# Autodesk Inventor assembly: Combined OmniWheel
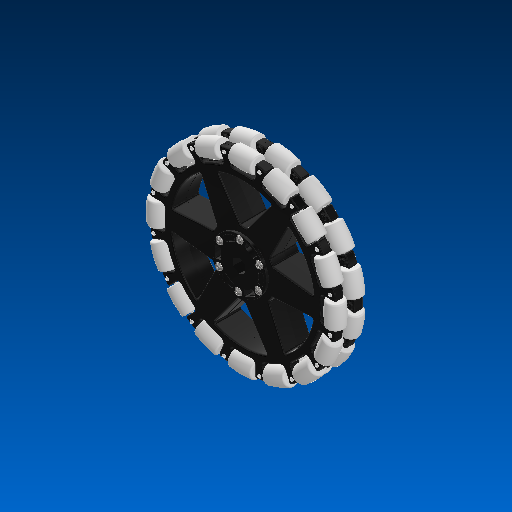
[picture p0: Inventor's stored thumbnail of the model, 512x512]
Saved by Autodesk Inventor 2022.2 (Build 262287000, 287)
## iProperties
Created: 2022-01-02
Part Number: Combined OmniWheel
Document SubType Name: Assembly
Designer: omard
Author: omard
## Documents named in this file (4)
- D:\omard\OneDrive - Auburn University\BasketBall Shooting Robot\Combined OmniWheel.iam
- D:\omard\OneDrive - Auburn University\BasketBall Shooting Robot\VEX Parts\1_2” Hex Bore Aluminum VersaHub (217-2592).ipt
- D:\omard\OneDrive - Auburn University\BasketBall Shooting Robot\VEX Parts\8 Omni-Directional Wheel (217-2613).iam
- D:\omard\OneDrive - Auburn University\BasketBall Shooting Robot\VEX Parts\#8-32 x 0.625 Star Drive Screw (276-4993).ipt
## Components (15 placed, 3 different names)
1. 1_2” Hex Bore Aluminum VersaHub (217-2592):1 — Mate:1, Mate:2, Mate:3, Angle:1, Mate:19, Mate:20, Mate:21, Mate:22, Mate:23, Mate:24, Mate:25, Mate:26, Mate:27, Mate:28, Mate:29, Mate:30
2. 8 Omni-Directional Wheel (217-2613):1 [sub-assembly] — Mate:1, Mate:2, Mate:3, Angle:1, Angle:2, Mate:4, Mate:5, Mate:6
3. 1_2” Hex Bore Aluminum VersaHub (217-2592):2 — Angle:2, Mate:4, Mate:5, Mate:6, Mate:7, Mate:8, Mate:9, Mate:10, Mate:11, Mate:12, Mate:13, Mate:14, Mate:15, Mate:16, Mate:17, Mate:18
4. #8-32 x 0.625 Star Drive Screw (276-4993):1 — Mate:7, Mate:14
5. #8-32 x 0.625 Star Drive Screw (276-4993):2 — Mate:12, Mate:13
6. #8-32 x 0.625 Star Drive Screw (276-4993):3 — Mate:11, Mate:18
7. #8-32 x 0.625 Star Drive Screw (276-4993):4 — Mate:10, Mate:17
8. #8-32 x 0.625 Star Drive Screw (276-4993):5 — Mate:9, Mate:16
9. #8-32 x 0.625 Star Drive Screw (276-4993):6 — Mate:8, Mate:15
10. #8-32 x 0.625 Star Drive Screw (276-4993):7 — Mate:25, Mate:30
11. #8-32 x 0.625 Star Drive Screw (276-4993):8 — Mate:24, Mate:29
12. #8-32 x 0.625 Star Drive Screw (276-4993):9 — Mate:23, Mate:28
13. #8-32 x 0.625 Star Drive Screw (276-4993):10 — Mate:22, Mate:27
14. #8-32 x 0.625 Star Drive Screw (276-4993):11 — Mate:19, Mate:20
15. #8-32 x 0.625 Star Drive Screw (276-4993):12 — Mate:21, Mate:26
## Relationships (32: Mate 30, Angle 2)
- Mate:1: 1_2” Hex Bore Aluminum VersaHub (217-2592):1 ↔ 8 Omni-Directional Wheel (217-2613):1
- Mate:2: 1_2” Hex Bore Aluminum VersaHub (217-2592):1 ↔ 8 Omni-Directional Wheel (217-2613):1
- Mate:3: 1_2” Hex Bore Aluminum VersaHub (217-2592):1 ↔ 8 Omni-Directional Wheel (217-2613):1
- Angle:1 (0 deg): 1_2” Hex Bore Aluminum VersaHub (217-2592):1 ↔ 8 Omni-Directional Wheel (217-2613):1
- Angle:2 (0 deg): 8 Omni-Directional Wheel (217-2613):1 ↔ 1_2” Hex Bore Aluminum VersaHub (217-2592):2
- Mate:4: 8 Omni-Directional Wheel (217-2613):1 ↔ 1_2” Hex Bore Aluminum VersaHub (217-2592):2
- Mate:5: 8 Omni-Directional Wheel (217-2613):1 ↔ 1_2” Hex Bore Aluminum VersaHub (217-2592):2
- Mate:6: 8 Omni-Directional Wheel (217-2613):1 ↔ 1_2” Hex Bore Aluminum VersaHub (217-2592):2
- Mate:7: 1_2” Hex Bore Aluminum VersaHub (217-2592):2 ↔ #8-32 x 0.625 Star Drive Screw (276-4993):1
- Mate:8: 1_2” Hex Bore Aluminum VersaHub (217-2592):2 ↔ #8-32 x 0.625 Star Drive Screw (276-4993):6
- Mate:9: 1_2” Hex Bore Aluminum VersaHub (217-2592):2 ↔ #8-32 x 0.625 Star Drive Screw (276-4993):5
- Mate:10: 1_2” Hex Bore Aluminum VersaHub (217-2592):2 ↔ #8-32 x 0.625 Star Drive Screw (276-4993):4
- Mate:11: 1_2” Hex Bore Aluminum VersaHub (217-2592):2 ↔ #8-32 x 0.625 Star Drive Screw (276-4993):3
- Mate:12: 1_2” Hex Bore Aluminum VersaHub (217-2592):2 ↔ #8-32 x 0.625 Star Drive Screw (276-4993):2
- Mate:13: 1_2” Hex Bore Aluminum VersaHub (217-2592):2 ↔ #8-32 x 0.625 Star Drive Screw (276-4993):2
- Mate:14: 1_2” Hex Bore Aluminum VersaHub (217-2592):2 ↔ #8-32 x 0.625 Star Drive Screw (276-4993):1
- Mate:15: 1_2” Hex Bore Aluminum VersaHub (217-2592):2 ↔ #8-32 x 0.625 Star Drive Screw (276-4993):6
- Mate:16: 1_2” Hex Bore Aluminum VersaHub (217-2592):2 ↔ #8-32 x 0.625 Star Drive Screw (276-4993):5
- Mate:17: 1_2” Hex Bore Aluminum VersaHub (217-2592):2 ↔ #8-32 x 0.625 Star Drive Screw (276-4993):4
- Mate:18: 1_2” Hex Bore Aluminum VersaHub (217-2592):2 ↔ #8-32 x 0.625 Star Drive Screw (276-4993):3
- Mate:19: 1_2” Hex Bore Aluminum VersaHub (217-2592):1 ↔ #8-32 x 0.625 Star Drive Screw (276-4993):11
- Mate:20: 1_2” Hex Bore Aluminum VersaHub (217-2592):1 ↔ #8-32 x 0.625 Star Drive Screw (276-4993):11
- Mate:21: 1_2” Hex Bore Aluminum VersaHub (217-2592):1 ↔ #8-32 x 0.625 Star Drive Screw (276-4993):12
- Mate:22: 1_2” Hex Bore Aluminum VersaHub (217-2592):1 ↔ #8-32 x 0.625 Star Drive Screw (276-4993):10
- Mate:23: 1_2” Hex Bore Aluminum VersaHub (217-2592):1 ↔ #8-32 x 0.625 Star Drive Screw (276-4993):9
- Mate:24: 1_2” Hex Bore Aluminum VersaHub (217-2592):1 ↔ #8-32 x 0.625 Star Drive Screw (276-4993):8
- Mate:25: 1_2” Hex Bore Aluminum VersaHub (217-2592):1 ↔ #8-32 x 0.625 Star Drive Screw (276-4993):7
- Mate:26: 1_2” Hex Bore Aluminum VersaHub (217-2592):1 ↔ #8-32 x 0.625 Star Drive Screw (276-4993):12
- Mate:27: 1_2” Hex Bore Aluminum VersaHub (217-2592):1 ↔ #8-32 x 0.625 Star Drive Screw (276-4993):10
- Mate:28: 1_2” Hex Bore Aluminum VersaHub (217-2592):1 ↔ #8-32 x 0.625 Star Drive Screw (276-4993):9
- Mate:29: 1_2” Hex Bore Aluminum VersaHub (217-2592):1 ↔ #8-32 x 0.625 Star Drive Screw (276-4993):8
- Mate:30: 1_2” Hex Bore Aluminum VersaHub (217-2592):1 ↔ #8-32 x 0.625 Star Drive Screw (276-4993):7
